# Autodesk Inventor assembly: 4 in HiGrip Wheel
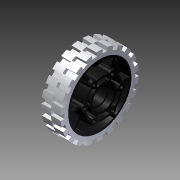
[picture p0: Inventor's stored thumbnail of the model, 180x180]
Saved by Autodesk Inventor 2012 (Build 160160000, 160)
## iProperties
Created: 2013-07-13
Part Number: 4 in HiGrip Wheel
Document SubType Name: Assembly
Designer: Bryce
Author: Bryce
Translation Standard: STEP AP203
FileName: 4 in HiGrip Wheel.STEP
PreProcessor: SolidWorks 2010
PostProcessor: Build: 160, Release: 2012 RTM - Date: Tue 03/01/2011
Sent Units: inch
Uncertainty: 1e-05
## Documents named in this file (3)
- C:\Users\Bryce\Dropbox\Inventor Design Project Files\Independent Swerves\Imported Components\4 in HiGrip Wheel\4 in HiGrip Wheel.iam
- C:\Users\Bryce\Dropbox\Inventor Design Project Files\Independent Swerves\Imported Components\4 in HiGrip Wheel\4 in tread.ipt
- C:\Users\Bryce\Dropbox\Inventor Design Project Files\Independent Swerves\Imported Components\4 in HiGrip Wheel\4in 2013 Hub.ipt
## Components (2 placed, 2 different names)
1. 4 in tread:1 — Mate:1, Flush:1
2. 4in 2013 Hub:1 — Mate:1, Flush:1
## Relationships (2: Mate 1, Flush 1)
- Mate:1: 4 in tread:1 ↔ 4in 2013 Hub:1
- Flush:1: 4 in tread:1 ↔ 4in 2013 Hub:1
